# Autodesk Inventor assembly: Assembly1
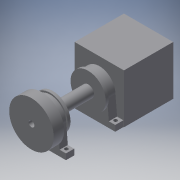
[picture p0: Inventor's stored thumbnail of the model, 180x180]
Saved by Autodesk Inventor 2017 (Build 210142000, 142)
## iProperties
Created: 2017-04-28
Part Number: Assembly1
Document SubType Name: Assembly
Designer: s4321966
Author: s4321966
## Documents named in this file (6)
- \\puffball.labs.eait.uq.edu.au\s4321966\Documents\metr4810_spool draft\Assembly1.iam
- \\puffball.labs.eait.uq.edu.au\s4321966\Documents\metr4810_spool draft\nema17.ipt
- \\puffball.labs.eait.uq.edu.au\s4321966\Documents\metr4810_spool draft\spool.ipt
- \\puffball.labs.eait.uq.edu.au\s4321966\Documents\metr4810_spool draft\std_bearing.ipt
- \\puffball.labs.eait.uq.edu.au\s4321966\Documents\metr4810_spool draft\mount.ipt
- \\puffball.labs.eait.uq.edu.au\s4321966\Documents\metr4810_spool draft\slipring.ipt
## Components (7 placed, 5 different names)
1. nema17:1 — Rotational:1, Flush:3, Flush:4
2. spool:1 — Cylindrical:1, Flush:1, Cylindrical:2, Flush:2, Mate:1, Mate:2, Cylindrical:5
3. std_bearing:1 — Cylindrical:1, Flush:1, Cylindrical:3
4. std_bearing:2 — Cylindrical:2, Flush:2, Rotational:1, Cylindrical:4
5. mount:1 — Flush:4, Cylindrical:3, Mate:1, Mate:3
6. mount:2 — Flush:3, Cylindrical:4, Mate:2
7. slipring:1 — Mate:3, Cylindrical:5
## Relationships (13: CylindricalJoint 5, Flush 4, Mate 3, RevoluteJoint 1)
- Cylindrical:1: spool:1 ↔ std_bearing:1
- Flush:1: spool:1 ↔ std_bearing:1
- Cylindrical:2: spool:1 ↔ std_bearing:2
- Flush:2: spool:1 ↔ std_bearing:2
- Rotational:1 [RevoluteJoint]: nema17:1 ↔ std_bearing:2
- Flush:3: nema17:1 ↔ mount:2
- Flush:4: nema17:1 ↔ mount:1
- Cylindrical:3: std_bearing:1 ↔ mount:1
- Cylindrical:4: std_bearing:2 ↔ mount:2
- Mate:1: spool:1 ↔ mount:1
- Mate:2: spool:1 ↔ mount:2
- Mate:3: mount:1 ↔ slipring:1
- Cylindrical:5: spool:1 ↔ slipring:1
